# Autodesk Inventor assembly: GE-13028
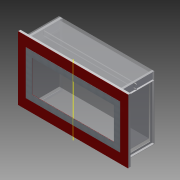
[picture p0: Inventor's stored thumbnail of the model, 180x180]
Saved by Autodesk Inventor 2013 (Build 170138000, 138)
## iProperties
Created: 2013-01-04
Part Number: GE-13028
Document SubType Name: Assembly
Designer: Phillip
Author: Phillip
## Documents named in this file (10)
- C:\Users\Moses\Documents\Inventor\2013 Team 3061 Robot\FIRST Arena 2013\Feeder Goal Station\GE-13028.iam
- C:\Users\Moses\Documents\Inventor\2013 Team 3061 Robot\FIRST Arena 2013\Feeder Goal Station\GE-13062.iam
- C:\Users\Moses\Documents\Inventor\2013 Team 3061 Robot\FIRST Arena 2013\Feeder Goal Station\GE-13029.ipt
- C:\Users\Moses\Documents\Inventor\2013 Team 3061 Robot\FIRST Arena 2013\Feeder Goal Station\GE_13030.ipt
- C:\Users\Moses\Documents\Inventor\2013 Team 3061 Robot\FIRST Arena 2013\Feeder Goal Station\box_middlegoal.ipt
- C:\Users\Moses\Documents\Inventor\2013 Team 3061 Robot\FIRST Arena 2013\Feeder Goal Station\GE-13011B.ipt
- C:\Users\Moses\Documents\Inventor\2013 Team 3061 Robot\FIRST Arena 2013\Feeder Goal Station\GE-13061.iam
- C:\Users\Moses\Documents\Inventor\2013 Team 3061 Robot\FIRST Arena 2013\Feeder Goal Station\GE-13031.ipt
- C:\Users\Moses\Documents\Inventor\2013 Team 3061 Robot\FIRST Arena 2013\Feeder Goal Station\GE-13064.ipt
- C:\Users\Moses\Documents\Inventor\2013 Team 3061 Robot\FIRST Arena 2013\Feeder Goal Station\Reflective02.ipt
## Components (11 placed, 9 different names)
1. GE-13062:1 [sub-assembly] — Mate:1, Angle:1, Flush:1, Mate:2, Flush:2, Mate:4, Mate:7, Mate:14, Mate:15, Mate:16, Mate:23
2. GE-13029:1 — Mate:24, Flush:4, Flush:5
3. GE_13030:1 — Mate:9, Mate:11, Mate:13, Mate:24, Flush:4, Mate:25
4. GE_13030:2 — Mate:20, Mate:21, Mate:22
5. box_middlegoal:1 — Mate:1, Angle:1, Mate:3, Mate:6, Mate:19
6. GE-13011B:1 — Flush:1, Mate:2, Flush:2, Flush:6, Flush:7, Mate:26, Angle:2
7. GE-13061:1 [sub-assembly] — Mate:3, Mate:4, Mate:9, Mate:11, Mate:13, Flush:3, Mate:17
8. GE-13061:2 [sub-assembly] — Mate:6, Mate:7, Mate:18, Mate:20, Mate:21, Mate:22, Mate:23
9. GE-13031:1 — Mate:14, Mate:15, Mate:16, Flush:3, Mate:17, Mate:18, Mate:19
10. GE-13064:1 — Mate:25, Flush:5
11. Reflective02:1 — Flush:6, Flush:7
## Relationships (31: Mate 22, Flush 7, Angle 2)
- Mate:1: GE-13062:1 ↔ box_middlegoal:1
- Angle:1 (0 deg): GE-13062:1 ↔ box_middlegoal:1
- Flush:1: GE-13062:1 ↔ GE-13011B:1
- Mate:2: GE-13062:1 ↔ GE-13011B:1
- Flush:2: GE-13062:1 ↔ GE-13011B:1
- Mate:3: box_middlegoal:1 ↔ GE-13061:1
- Mate:4: GE-13062:1 ↔ GE-13061:1
- Mate:6: box_middlegoal:1 ↔ GE-13061:2
- Mate:7: GE-13062:1 ↔ GE-13061:2
- Mate:9: GE_13030:1 ↔ GE-13061:1
- Mate:11: GE_13030:1 ↔ GE-13061:1
- Mate:13: GE_13030:1 ↔ GE-13061:1
- Mate:14: GE-13062:1 ↔ GE-13031:1
- Mate:15: GE-13062:1 ↔ GE-13031:1
- Mate:16: GE-13062:1 ↔ GE-13031:1
- Flush:3: GE-13061:1 ↔ GE-13031:1
- Mate:17: GE-13061:1 ↔ GE-13031:1
- Mate:18: GE-13061:2 ↔ GE-13031:1
- Mate:19: box_middlegoal:1 ↔ GE-13031:1
- Mate:20: GE_13030:2 ↔ GE-13061:2
- Mate:21: GE_13030:2 ↔ GE-13061:2
- Mate:22: GE_13030:2 ↔ GE-13061:2
- Mate:23 (133.35 mm): GE-13062:1 ↔ GE-13061:2
- Mate:24: GE-13029:1 ↔ GE_13030:1
- Flush:4 (33.3375 mm): GE-13029:1 ↔ GE_13030:1
- Mate:25: GE_13030:1 ↔ GE-13064:1
- Flush:5: GE-13029:1 ↔ GE-13064:1
- Flush:6: GE-13011B:1 ↔ Reflective02:1
- Flush:7: GE-13011B:1 ↔ Reflective02:1
- Mate:26: GE-13011B:1
- Angle:2 (0 deg): GE-13011B:1
